# Autodesk Inventor assembly: XM,H-430_idler
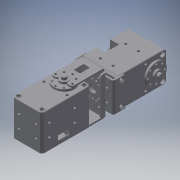
[picture p0: Inventor's stored thumbnail of the model, 180x180]
Saved by Autodesk Inventor 2019 (Build 230136000, 136)
## iProperties
Created: 2016-05-16
Part Number: XM,H-430_idler
Material: 일반
Document SubType Name: Assembly
Designer: bong
Title: X-430_IDLE_20160516_ASM
Author: RICK
Revision Number: 5LAST_VERSION
Sending System: PRO/ENGINEER BY PARAMETRIC TECHNOLOGY CORPORATION, 2013410
Preprocessor: PRO/ENGINEER BY PARAMETRIC TECHNOLOGY CORPORATION, 2013410
## Documents named in this file (6)
- C:\Users\bong\project\snake_RL\description\XM,H-430_idler.iam
- C:\Users\bong\project\snake_RL\description\X-430_IDLE.ipt
- C:\Users\bong\project\snake_RL\description\X-430_SPACER_RING.ipt
- C:\Users\bong\project\snake_RL\description\X-430_CVR_CABLE.ipt
- C:\Users\bong\project\snake_RL\description\fr12_h101.ipt
- C:\Users\bong\project\snake_RL\description\fr12_s102.ipt
## Components (13 placed, 13 different names)
1. X-430_IDLE_10 — 메이트:1, 메이트:2, 메이트:3
2. X-430_SPACER_RING_11
3. X-430_SPACER_RING_12
4. X-430_SPACER_RING_13
5. X-430_SPACER_RING_14
6. X-430_SPACER_RING_15
7. X-430_SPACER_RING_16
8. X-430_SPACER_RING_17
9. X-430_SPACER_RING_18
10. X-430_CVR_CABLE_19
11. fr12_h101:1 — 메이트:1, 메이트:2, 메이트:3, 메이트:4, 메이트:5, 메이트:6
12. fr12_s102:1 — 메이트:4, 메이트:5, 메이트:6, 메이트:7, 메이트:8, 메이트:9
13. X-430_IDLE:2 — 메이트:7, 메이트:8, 메이트:9
## Relationships (9: Mate 9)
- 메이트:1 [Mate]: X-430_IDLE_10 ↔ fr12_h101:1
- 메이트:2 [Mate]: X-430_IDLE_10 ↔ fr12_h101:1
- 메이트:3 [Mate]: X-430_IDLE_10 ↔ fr12_h101:1
- 메이트:4 [Mate]: fr12_h101:1 ↔ fr12_s102:1
- 메이트:5 [Mate]: fr12_h101:1 ↔ fr12_s102:1
- 메이트:6 [Mate]: fr12_h101:1 ↔ fr12_s102:1
- 메이트:7 [Mate]: fr12_s102:1 ↔ X-430_IDLE:2
- 메이트:8 [Mate]: fr12_s102:1 ↔ X-430_IDLE:2
- 메이트:9 [Mate]: fr12_s102:1 ↔ X-430_IDLE:2
